# Autodesk Inventor assembly: AssembledOnSmall
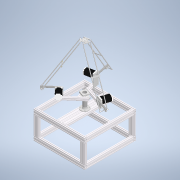
[picture p0: Inventor's stored thumbnail of the model, 180x180]
Saved by Autodesk Inventor 2021 (Build 250183000, 183)
## iProperties
Created: 2022-09-12
Part Number: AssembledOnSmall
Document SubType Name: Assembly
Designer: szucs
Author: szucs
## Documents named in this file (3)
- C:\Git\PhD\Inventor\GTPR_toBeBuilt\AssembledOnSmall.iam
- C:\Git\PhD\Inventor\GTPR_toBeBuilt\mount\mount_small.iam
- C:\Git\PhD\Inventor\GTPR_toBeBuilt\GTPR Assembly - Laci.iam
## Components (2 placed, 2 different names)
1. mount_small:1 [sub-assembly] — Mate:1, Mate:2, Mate:3, Angle:1
2. GTPR Assembly - Laci:1 [sub-assembly] — Mate:1, Mate:2, Mate:3, Angle:1
## Relationships (4: Mate 3, Angle 1)
- Mate:1: mount_small:1 ↔ GTPR Assembly - Laci:1
- Mate:2 (-425 mm): mount_small:1 ↔ GTPR Assembly - Laci:1
- Mate:3 (-425 mm): mount_small:1 ↔ GTPR Assembly - Laci:1
- Angle:1 (0 deg): mount_small:1 ↔ GTPR Assembly - Laci:1
